# Autodesk Inventor assembly: PIXYWITHRING
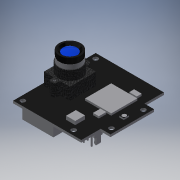
[picture p0: Inventor's stored thumbnail of the model, 180x180]
Saved by Autodesk Inventor 2017 (Build 210142000, 142)
## iProperties
Created: 2016-12-19
Part Number: PIXYWITHRING
Document SubType Name: Assembly
Designer: PLTW
Author: PLTW
## Documents named in this file (3)
- C:\Users\PLTW\Documents\Inventor\PixyCam and Gimbal\PIXYWITHRING.iam
- C:\Users\PLTW\Documents\Inventor\PixyCam and Gimbal\PixyCamKinda.ipt
- C:\Users\PLTW\Documents\Inventor\PixyCam and Gimbal\focusSpacer.ipt
## Components (2 placed, 2 different names)
1. PixyCamKinda:1 — Flush:1
2. focusSpacer:1 — Flush:1
## Relationships (1: Flush 1)
- Flush:1: PixyCamKinda:1 ↔ focusSpacer:1
